# Autodesk Inventor assembly: tempAsm
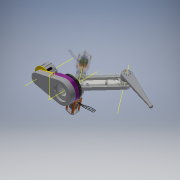
[picture p0: Inventor's stored thumbnail of the model, 180x180]
Saved by Autodesk Inventor 2018 (Build 220112000, 112)
## iProperties
Created: 2020-03-07
Part Number: tempAsm
Document SubType Name: Assembly
Designer: Bunny320
Author: Bunny320
## Documents named in this file (5)
- C:\Users\Bunny320\Desktop\sechs\4-CAD\tempAsm.iam
- C:\Users\Bunny320\Desktop\sechs\4-CAD\10-J1.iam
- C:\Users\Bunny320\Desktop\sechs\4-CAD\20-J2.iam
- C:\Users\Bunny320\Desktop\sechs\4-CAD\30-J3.iam
- C:\Users\Bunny320\Desktop\sechs\4-CAD\J4-dummy.ipt
## Components (4 placed, 4 different names)
1. 10-J1:1 [sub-assembly] — Flush:1, Flush:2, Flush:3, Mate:1, Mate:2, Mate:3, Mate:4, Mate:5, Mate:6
2. 20-J2:1 [sub-assembly] — Mate:1, Mate:2, Mate:3, Flush:4
3. 30-J3:1 [sub-assembly] — Mate:4, Mate:5, Mate:6, Flush:4, Mate:7, Mate:8
4. J4-dummy:1 — Mate:7, Mate:8
## Relationships (12: Mate 8, Flush 4)
- Flush:1: 10-J1:1
- Flush:2: 10-J1:1
- Flush:3: 10-J1:1
- Mate:1: 10-J1:1 ↔ 20-J2:1
- Mate:2: 10-J1:1 ↔ 20-J2:1
- Mate:3: 10-J1:1 ↔ 20-J2:1
- Mate:4: 10-J1:1 ↔ 30-J3:1
- Mate:5: 10-J1:1 ↔ 30-J3:1
- Mate:6: 10-J1:1 ↔ 30-J3:1
- Flush:4: 20-J2:1 ↔ 30-J3:1
- Mate:7: 30-J3:1 ↔ J4-dummy:1
- Mate:8: 30-J3:1 ↔ J4-dummy:1
